# Autodesk Inventor assembly: slopeAssembly
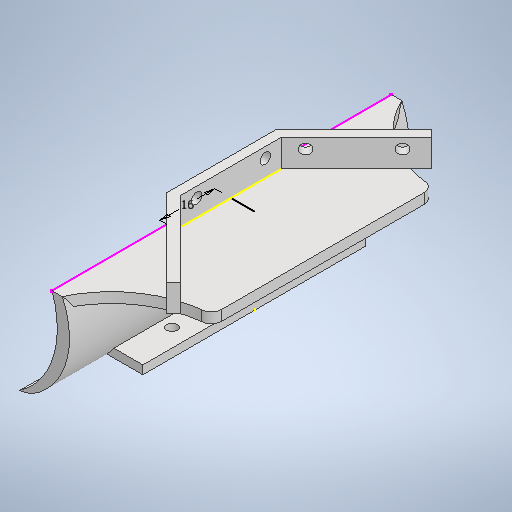
[picture p0: Inventor's stored thumbnail of the model, 512x512]
Saved by Autodesk Inventor 2025.1 (Build 291241020, 241B)
## iProperties
Created: 2025-04-16
Part Number: slopeAssembly
Document SubType Name: Assembly
Designer: omiye
Author: omiye
## Documents named in this file (3)
- C:\Projects\Arduino\sumobotV2\models\slopeAssembly.iam
- C:\Projects\Arduino\sumobotV2\models\slope.ipt
- C:\Projects\Arduino\sumobotV2\models\distanceSensorMountIncl.ipt
## Components (2 placed, 2 different names)
1. slope:1 — Mate:1, Mate:8, Mate:9
2. distanceSensorMountIncl:1 — Mate:1, Mate:8, Mate:9
## Relationships (3: Mate 3)
- Mate:1: slope:1 ↔ distanceSensorMountIncl:1
- Mate:8: slope:1 ↔ distanceSensorMountIncl:1
- Mate:9: slope:1 ↔ distanceSensorMountIncl:1
